# Autodesk Inventor assembly: upper_chassis
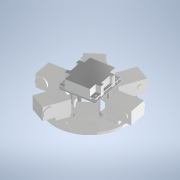
[picture p0: Inventor's stored thumbnail of the model, 180x180]
Saved by Autodesk Inventor 2020.2 (Build 242310000, 310)
## iProperties
Created: 2020-11-22
Part Number: upper_chassis
Document SubType Name: Assembly
Designer: mazzo
Author: mazzo
## Documents named in this file (5)
- D:\Documenti\università\Progetto Meccanica dei Robot\assembled in urdf\upper_chassis.iam
- D:\Documenti\università\Progetto Meccanica dei Robot\meccanica\parti autodesk\V6\V6 Luca\OpenCM485EXP.ipt
- D:\Documenti\università\Progetto Meccanica dei Robot\meccanica\parti autodesk\V6\V6 Luca\upper_chassis.ipt
- D:\Documenti\università\Progetto Meccanica dei Robot\meccanica\parti autodesk\V6\V6 Luca\upper_chassis_holder_v2.ipt
- D:\Documenti\università\Progetto Meccanica dei Robot\meccanica\parti autodesk\V6\V6 Luca\Motore2.ipt
## Components (9 placed, 4 different names)
1. OpenCM485EXP:1 — Coincidente:6, Coincidente:7, Coincidente:8
2. upper_chassis:1 — Coincidente:1, Coincidente:2, Coincidente:3, Coincidente:4, Coincidente:5, Coincidente:9, Coincidente:10, Coincidente:11
3. upper_chassis_holder_v2:1 — Coincidente:3, Coincidente:4, Coincidente:5, Coincidente:6, Coincidente:7, Coincidente:8
4. Motore2:1 — Coincidente:9, Coincidente:10, Coincidente:11
5. Motore2:2
6. Motore2:3
7. Motore2:4
8. Motore2:5
9. Motore2:6
## Component patterns: (6 elements, first: Motore2:1)
## Relationships (11: Mate 11)
- Coincidente:1 [Mate]: upper_chassis:1
- Coincidente:2 [Mate]: upper_chassis:1
- Coincidente:3 [Mate]: upper_chassis:1 ↔ upper_chassis_holder_v2:1
- Coincidente:4 [Mate]: upper_chassis:1 ↔ upper_chassis_holder_v2:1
- Coincidente:5 [Mate]: upper_chassis:1 ↔ upper_chassis_holder_v2:1
- Coincidente:6 [Mate]: OpenCM485EXP:1 ↔ upper_chassis_holder_v2:1
- Coincidente:7 [Mate]: OpenCM485EXP:1 ↔ upper_chassis_holder_v2:1
- Coincidente:8 [Mate]: OpenCM485EXP:1 ↔ upper_chassis_holder_v2:1
- Coincidente:9 [Mate]: upper_chassis:1 ↔ Motore2:1
- Coincidente:10 [Mate]: upper_chassis:1 ↔ Motore2:1
- Coincidente:11 [Mate]: upper_chassis:1 ↔ Motore2:1
